# Autodesk Inventor assembly: RobotV1
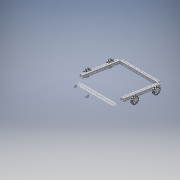
[picture p0: Inventor's stored thumbnail of the model, 180x180]
Saved by Autodesk Inventor 2017 (Build 210142000, 142)
## iProperties
Created: 2017-09-13
Part Number: RobotV1
Document SubType Name: Assembly
Designer: Kenneth
Author: Kenneth
## Documents named in this file (8)
- C:\Workspaces\CAD\RobotV1.iam
- C:\Workspaces\CAD\Spectrum-CAD-Library\FTC\FTC Tetrix KOP\Channel 416mm.ipt
- C:\Workspaces\CAD\Spectrum-CAD-Library\FTC\FTC Tetrix KOP\Bracket L-angle.ipt
- C:\Workspaces\CAD\Spectrum-CAD-Library\FTC\FTC Tetrix KOP\Bearing Flange 3mm x 4mm x 8mm.ipt
- C:\Workspaces\CAD\Spectrum-CAD-Library\FTC\FTC Tetrix KOP\Axle 100mm.ipt
- C:\Workspaces\CAD\Spectrum-CAD-Library\FTC\FTC Tetrix KOP\Axle Shaft Hub.ipt
- C:\Workspaces\CAD\Spectrum-CAD-Library\FTC\FTC Tetrix KOP\Omni Wheel 3 inch.ipt
- C:\Workspaces\CAD\Spectrum-CAD-Library\FTC\FTC Tetrix KOP\Omni Wheel Joining Ring.ipt
## Components (32 placed, 7 different names)
1. Channel 416mm:1 — Mate:8, Mate:10, Mate:11, Mate:33, Mate:34, Mate:35, Mate:36
2. Channel 416mm:2 — Mate:15, Mate:16, Mate:17, Mate:37, Mate:38, Mate:39, Mate:40
3. Channel 416mm:3 — Mate:2, Mate:4, Mate:5, Mate:93
4. Channel 416mm:4 — Mate:7, Mate:9, Mate:12, Mate:13, Mate:14, Mate:18
5. Bracket L-angle:1 — Mate:2, Mate:4, Mate:5, Mate:93
6. Bracket L-angle:2
7. Bracket L-angle:3 — Mate:7, Mate:8, Mate:9, Mate:10, Mate:11, Mate:12
8. Bracket L-angle:4 — Mate:13, Mate:14, Mate:15, Mate:16, Mate:17, Mate:18
9. Bearing Flange 3mm x 4mm x 8mm:1 — Mate:35, Mate:36, Mate:43
10. Bearing Flange 3mm x 4mm x 8mm:2 — Mate:33, Mate:34, Mate:44
11. Bearing Flange 3mm x 4mm x 8mm:3 — Mate:37, Mate:38, Mate:42
12. Bearing Flange 3mm x 4mm x 8mm:4 — Mate:39, Mate:40, Mate:41
13. Axle 100mm:1 — Mate:41, Mate:53, Mate:87
14. Axle 100mm:2 — Mate:42, Mate:54, Mate:84
15. Axle 100mm:3 — Mate:44, Mate:56, Mate:90
16. Axle 100mm:4 — Mate:43, Mate:55, Mate:81
17. Axle Shaft Hub:1 — Mate:53, Mate:88, Mate:89
18. Axle Shaft Hub:2 — Mate:54, Mate:85, Mate:86
19. Axle Shaft Hub:3 — Mate:56, Mate:91, Mate:92
20. Axle Shaft Hub:4 — Mate:55, Mate:82, Mate:83
21. Omni Wheel 3 inch:3 — Mate:90, Mate:91, Mate:92
22. Omni Wheel 3 inch:4
23. Omni Wheel Joining Ring:2
24. Omni Wheel 3 inch:5
25. Omni Wheel 3 inch:6 — Mate:87, Mate:88, Mate:89
26. Omni Wheel Joining Ring:3
27. Omni Wheel 3 inch:7
28. Omni Wheel 3 inch:8 — Mate:84, Mate:85, Mate:86
29. Omni Wheel Joining Ring:4
30. Omni Wheel 3 inch:1 — Mate:57, Mate:58, Mate:59, Mate:82, Mate:83
31. Omni Wheel 3 inch:2 — Mate:60, Mate:61, Mate:62, Mate:81
32. Omni Wheel Joining Ring:1 — Mate:57, Mate:58, Mate:59, Mate:60, Mate:61, Mate:62
## Relationships (68: Mate 68)
- Mate:2: Channel 416mm:3 ↔ Bracket L-angle:1
- Mate:4: Channel 416mm:3 ↔ Bracket L-angle:1
- Mate:5: Channel 416mm:3 ↔ Bracket L-angle:1
- Mate:7: Channel 416mm:4 ↔ Bracket L-angle:3
- Mate:8: Channel 416mm:1 ↔ Bracket L-angle:3
- Mate:9: Channel 416mm:4 ↔ Bracket L-angle:3
- Mate:10: Channel 416mm:1 ↔ Bracket L-angle:3
- Mate:11: Channel 416mm:1 ↔ Bracket L-angle:3
- Mate:12: Channel 416mm:4 ↔ Bracket L-angle:3
- Mate:13: Channel 416mm:4 ↔ Bracket L-angle:4
- Mate:14: Channel 416mm:4 ↔ Bracket L-angle:4
- Mate:15: Channel 416mm:2 ↔ Bracket L-angle:4
- Mate:16: Channel 416mm:2 ↔ Bracket L-angle:4
- Mate:17: Channel 416mm:2 ↔ Bracket L-angle:4
- Mate:18: Channel 416mm:4 ↔ Bracket L-angle:4
- Mate:33: Channel 416mm:1 ↔ Bearing Flange 3mm x 4mm x 8mm:2
- Mate:34: Channel 416mm:1 ↔ Bearing Flange 3mm x 4mm x 8mm:2
- Mate:35: Channel 416mm:1 ↔ Bearing Flange 3mm x 4mm x 8mm:1
- Mate:36: Channel 416mm:1 ↔ Bearing Flange 3mm x 4mm x 8mm:1
- Mate:37: Channel 416mm:2 ↔ Bearing Flange 3mm x 4mm x 8mm:3
- Mate:38: Channel 416mm:2 ↔ Bearing Flange 3mm x 4mm x 8mm:3
- Mate:39: Channel 416mm:2 ↔ Bearing Flange 3mm x 4mm x 8mm:4
- Mate:40: Channel 416mm:2 ↔ Bearing Flange 3mm x 4mm x 8mm:4
- Mate:41: Bearing Flange 3mm x 4mm x 8mm:4 ↔ Axle 100mm:1
- Mate:42: Bearing Flange 3mm x 4mm x 8mm:3 ↔ Axle 100mm:2
- Mate:43: Bearing Flange 3mm x 4mm x 8mm:1 ↔ Axle 100mm:4
- Mate:44: Bearing Flange 3mm x 4mm x 8mm:2 ↔ Axle 100mm:3
- Mate:53: Axle 100mm:1 ↔ Axle Shaft Hub:1
- Mate:54: Axle 100mm:2 ↔ Axle Shaft Hub:2
- Mate:55: Axle 100mm:4 ↔ Axle Shaft Hub:4
- Mate:56: Axle 100mm:3 ↔ Axle Shaft Hub:3
- Mate:57: Omni Wheel 3 inch:1 ↔ Omni Wheel Joining Ring:1
- Mate:58: Omni Wheel 3 inch:1 ↔ Omni Wheel Joining Ring:1
- Mate:59: Omni Wheel 3 inch:1 ↔ Omni Wheel Joining Ring:1
- Mate:60: Omni Wheel 3 inch:2 ↔ Omni Wheel Joining Ring:1
- Mate:61: Omni Wheel 3 inch:2 ↔ Omni Wheel Joining Ring:1
- Mate:62: Omni Wheel 3 inch:2 ↔ Omni Wheel Joining Ring:1
- [Mate]: Omni Wheel 3 inch:3 ↔ Omni Wheel Joining Ring:2
- [Mate]: Omni Wheel 3 inch:3 ↔ Omni Wheel Joining Ring:2
- [Mate]: Omni Wheel 3 inch:3 ↔ Omni Wheel Joining Ring:2
- [Mate]: Omni Wheel 3 inch:4 ↔ Omni Wheel Joining Ring:2
- [Mate]: Omni Wheel 3 inch:4 ↔ Omni Wheel Joining Ring:2
- [Mate]: Omni Wheel 3 inch:4 ↔ Omni Wheel Joining Ring:2
- [Mate]: Omni Wheel 3 inch:5 ↔ Omni Wheel Joining Ring:3
- [Mate]: Omni Wheel 3 inch:5 ↔ Omni Wheel Joining Ring:3
- [Mate]: Omni Wheel 3 inch:5 ↔ Omni Wheel Joining Ring:3
- [Mate]: Omni Wheel 3 inch:6 ↔ Omni Wheel Joining Ring:3
- [Mate]: Omni Wheel 3 inch:6 ↔ Omni Wheel Joining Ring:3
- [Mate]: Omni Wheel 3 inch:6 ↔ Omni Wheel Joining Ring:3
- [Mate]: Omni Wheel 3 inch:7 ↔ Omni Wheel Joining Ring:4
- [Mate]: Omni Wheel 3 inch:7 ↔ Omni Wheel Joining Ring:4
- [Mate]: Omni Wheel 3 inch:7 ↔ Omni Wheel Joining Ring:4
- [Mate]: Omni Wheel 3 inch:8 ↔ Omni Wheel Joining Ring:4
- [Mate]: Omni Wheel 3 inch:8 ↔ Omni Wheel Joining Ring:4
- [Mate]: Omni Wheel 3 inch:8 ↔ Omni Wheel Joining Ring:4
- Mate:81: Axle 100mm:4 ↔ Omni Wheel 3 inch:2
- Mate:82: Axle Shaft Hub:4 ↔ Omni Wheel 3 inch:1
- Mate:83: Axle Shaft Hub:4 ↔ Omni Wheel 3 inch:1
- Mate:84: Axle 100mm:2 ↔ Omni Wheel 3 inch:8
- Mate:85: Axle Shaft Hub:2 ↔ Omni Wheel 3 inch:8
- Mate:86: Axle Shaft Hub:2 ↔ Omni Wheel 3 inch:8
- Mate:87: Axle 100mm:1 ↔ Omni Wheel 3 inch:6
- Mate:88: Axle Shaft Hub:1 ↔ Omni Wheel 3 inch:6
- Mate:89: Axle Shaft Hub:1 ↔ Omni Wheel 3 inch:6
- Mate:90: Axle 100mm:3 ↔ Omni Wheel 3 inch:3
- Mate:91: Axle Shaft Hub:3 ↔ Omni Wheel 3 inch:3
- Mate:92: Axle Shaft Hub:3 ↔ Omni Wheel 3 inch:3
- Mate:93: Channel 416mm:3 ↔ Bracket L-angle:1
## Named parameters: d64_d57 = 0 mm, d65_d58 = 0 mm, d66_d59 = 0 mm, d67_d60 = 0 mm, d68_d61 = 0 mm, d69_d63 = 0 mm, d70_d57 = 0 mm, d71_d58 = 0 mm, d72_d59 = 0 mm, d73_d60 = 0 mm, d74_d61 = 0 mm, d75_d63 = 0 mm, d76_d57 = 0 mm, d77_d58 = 0 mm, d78_d59 = 0 mm, d79_d60 = 0 mm, d80_d61 = 0 mm, d81_d63 = 0 mm
